# Autodesk Inventor assembly: actuator Assembly1
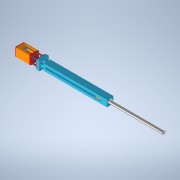
[picture p0: Inventor's stored thumbnail of the model, 180x180]
Saved by Autodesk Inventor 2021 (Build 250183000, 183)
## iProperties
Created: 2021-04-18
Part Number: actuator Assembly1
Document SubType Name: Assembly
Designer: ASUS
Author: ASUS
## Documents named in this file (10)
- E:\borewell rescuebot\pll manipulator files\sps manipulator\actuator Assembly1.iam
- E:\borewell rescuebot\pll manipulator files\sps manipulator\leadscrew.ipt
- E:\borewell rescuebot\pll manipulator files\sps manipulator\MicroGearmotor v3.ipt
- E:\borewell rescuebot\pll manipulator files\sps manipulator\plunger.ipt
- E:\borewell rescuebot\pll manipulator files\sps manipulator\piston.ipt
- E:\borewell rescuebot\pll manipulator files\sps manipulator\motor bracket n 20.ipt
- E:\borewell rescuebot\pll manipulator files\sps manipulator\female joint for uv.ipt
- E:\borewell rescuebot\pll manipulator files\sps manipulator\coupler.ipt
- E:\borewell rescuebot\pll manipulator files\sps manipulator\fab_model_mk-2[1]\Design Accelerator\Bearing1.iam
- E:\borewell rescuebot\pll manipulator files\sps manipulator\n20 motor 3dp support.ipt
## Components (9 placed, 9 different names)
1. leadscrew:1 — Rotation:1
2. MicroGearmotor v3:1 — Mate:10
3. plunger:1 — Rotation/Translation:1
4. piston:1 — Mate:11
5. motor bracket n 20:1 — Mate:11, Mate:12, Mate:13, Mate:14, Mate:15, Angle:4
6. female joint for uv:1 — Mate:13
7. coupler:1 — Mate:10, Mate:12, Rotation:1, Rotation/Translation:1
8. Bearing:1 [sub-assembly]
9. n20 motor 3dp support:1 — Mate:14, Mate:15, Angle:4, Mate:16, Mate:17
## Relationships (23: Mate 16, Angle 4, Flush 1, RelateRotation 1, RelateRotateTranslate 1)
- [Mate]: leadscrew:1 ↔ plunger:1
- [Angle] (0 deg): MicroGearmotor v3:1 ↔ motor bracket n 20:1
- [Mate]: motor bracket n 20:1 ↔ female joint for uv:1
- [Angle] (0 deg): piston:1 ↔ motor bracket n 20:1
- [Angle] (0 deg): plunger:1 ↔ piston:1
- [Mate]: piston:1 ↔ motor bracket n 20:1
- [Mate]: MicroGearmotor v3:1 ↔ motor bracket n 20:1
- [Mate]: leadscrew:1 ↔ MicroGearmotor v3:1
- [Mate]: leadscrew:1 ↔ Bearing:1
- [Flush]: motor bracket n 20:1 ↔ Bearing:1
- [Mate]: leadscrew:1 ↔ coupler:1
- [Mate]: coupler:1 ↔ Bearing:1
- Mate:10: MicroGearmotor v3:1 ↔ coupler:1
- Mate:11: piston:1 ↔ motor bracket n 20:1
- Mate:12: motor bracket n 20:1 ↔ coupler:1
- Mate:13: motor bracket n 20:1 ↔ female joint for uv:1
- Mate:14: motor bracket n 20:1 ↔ n20 motor 3dp support:1
- Mate:15: motor bracket n 20:1 ↔ n20 motor 3dp support:1
- Angle:4 (0 deg): motor bracket n 20:1 ↔ n20 motor 3dp support:1
- Rotation:1 [RelateRotation] (1 ul): leadscrew:1 ↔ coupler:1
- Rotation/Translation:1 [RelateRotateTranslate] (1 mm): plunger:1 ↔ coupler:1
- Mate:16: n20 motor 3dp support:1
- Mate:17: n20 motor 3dp support:1
